# Autodesk Inventor assembly: X roller assy
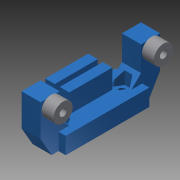
[picture p0: Inventor's stored thumbnail of the model, 180x180]
Saved by Autodesk Inventor 2013 (Build 170138000, 138)
## iProperties
Created: 2017-02-14
Part Number: X roller assy
Document SubType Name: Assembly
Designer: Herman de Vries
Author: Herman de Vries
## Documents named in this file (3)
- D:\Projects\Inventor\PaintBoid_2\X roller assy.iam
- D:\Projects\Inventor\PaintBoid_2\bearing 3mmx8mmx5mm.ipt
- D:\Projects\Inventor\PaintBoid_2\X rollers v2.ipt
## Components (3 placed, 2 different names)
1. X rollers v2:1 — Insert:1, Insert:2
2. bearing 3mmx10mmx5mm:1 — Insert:1
3. bearing 3mmx10mmx5mm:2 — Insert:2
## Relationships (2: Insert 2)
- Insert:1 (0.4 mm): X rollers v2:1 ↔ bearing 3mmx10mmx5mm:1
- Insert:2 (0.4 mm): X rollers v2:1 ↔ bearing 3mmx10mmx5mm:2
